# Autodesk Inventor assembly: 4138T531_Gas Spring (1)
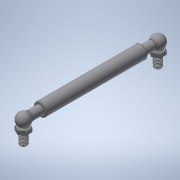
[picture p0: Inventor's stored thumbnail of the model, 180x180]
Saved by Autodesk Inventor 2020 (Build 240168000, 168)
## iProperties
Created: 2022-01-30
Part Number: 4138T531_Gas Spring (1)
Document SubType Name: Assembly
Designer: mavericks
Author: mavericks
## Documents named in this file (6)
- T:\EIT\2022 Rapid React\4138T531_Gas Spring (1).iam
- T:\EIT\2022 Rapid React\COMMON PARTS\MCMASTER\Gas spring\Solid1.ipt
- T:\EIT\2022 Rapid React\COMMON PARTS\MCMASTER\Gas spring\Solid2.ipt
- T:\EIT\2022 Rapid React\COMMON PARTS\MCMASTER\Gas spring\Solid3.ipt
- T:\EIT\2022 Rapid React\COMMON PARTS\MCMASTER\Gas spring\Solid4.ipt
- T:\EIT\2022 Rapid React\COMMON PARTS\MCMASTER\Gas spring\Solid7.ipt
## Components (5 placed, 5 different names)
1. Solid1:1
2. Solid2:1 — Angle:1, Mate:2
3. Solid3:1 — Mate:1, Tangent:1
4. Solid4:1 — Mate:1
5. Solid7:1 — Tangent:1, Angle:1, Mate:2
## Relationships (4: Mate 2, Tangent 1, Angle 1)
- Mate:1: Solid3:1 ↔ Solid4:1
- Tangent:1: Solid3:1 ↔ Solid7:1
- Angle:1 (0 deg): Solid2:1 ↔ Solid7:1
- Mate:2: Solid2:1 ↔ Solid7:1
